# Autodesk Inventor assembly: kamera_centre
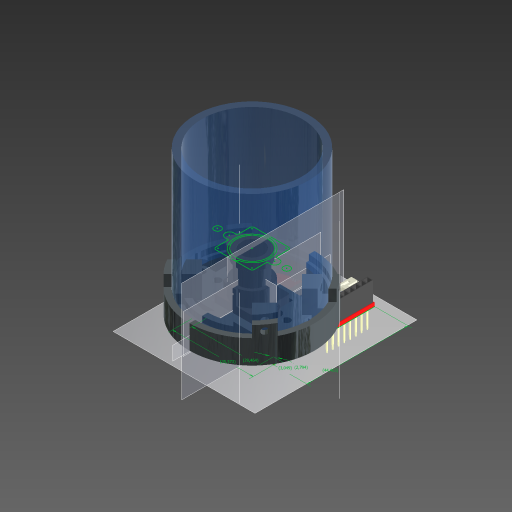
[picture p0: Inventor's stored thumbnail of the model, 512x512]
Saved by Autodesk Inventor 2023 (Build 270158000, 158)
## iProperties
Created: 2025-01-01
Part Number: kamera_centre
Document SubType Name: Assembly
Designer: Ivan
Mass: 38.1431 g
Surface Area: 427.9 cm^2
Volume: 36.4986 cm^3
Density: 1.04506 g/cm^3
Author: Ivan
## Documents named in this file (5)
- C:\Users\daa\Documents\DASH_V2\kamera_centre.iam
- C:\Users\daa\Documents\DASH_\Dash-V1\omv_centre.ipt
- C:\Users\daa\Documents\DASH_\Dash-V1\step\open_mv\openmv h7 plus alt.iam
- C:\Users\daa\Documents\DASH_\Dash-V1\t.ipt
- C:\Users\Ivan\Documents\Inventor\Content Center Files\R2020\ru-RU\Screw GOST R 1580-2013\Screw M3-6gx12 GOST R 50404-92(1).ipt
## Components (5 placed, 4 different names)
1. omv_centre:1 — Совмещение:1, Угол:1, Совмещение:2
2. openmv h7 plus alt:1 [sub-assembly] — Совмещение:1, Угол:1, Совмещение:2
3. t:1
4. Screw GOST R 1580-2013 M3-6gx12:1
5. Screw GOST R 1580-2013 M3-6gx12:2
## Relationships (3: Mate 2, Angle 1)
- Совмещение:1 [Mate]: omv_centre:1 ↔ openmv h7 plus alt:1
- Угол:1 [Angle] (180 deg): omv_centre:1 ↔ openmv h7 plus alt:1
- Совмещение:2 [Mate]: omv_centre:1 ↔ openmv h7 plus alt:1
